# Autodesk Inventor assembly: ASSEMBLY_Outlet_channel_1
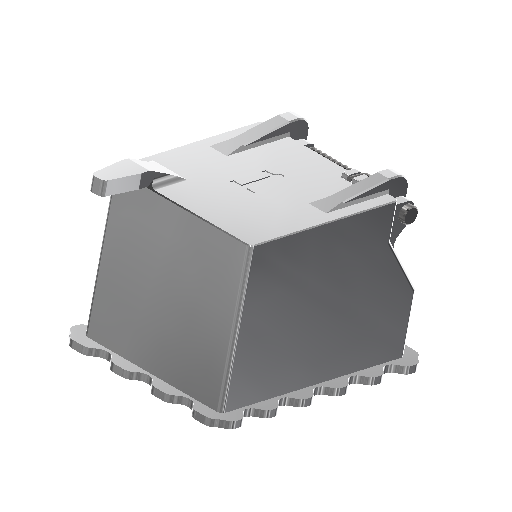
[picture p0: Inventor's stored thumbnail of the model, 512x512]
Saved by Autodesk Inventor 2025 (Build 290162010, 162A)
## iProperties
Created: 2018-09-15
Part Number: ASSEMBLY_Outlet_channel_1
Document SubType Name: Assembly
Designer: Andrzej
Mass: 26.9847 g
Surface Area: 139.625 cm^2
Volume: 9.56694 cm^3
Density: 2.82062 g/cm^3
Author: Andrzej
## Documents named in this file (5)
- D:\_ANDRZEJ_LACZEWSKI\_OTHER\MECH - My entry for the NASA Lunar Sampling System Design Challenge\MCAD\1_REV1\ASSEMBLY_MAIN_REVA\ASSEMBLY_Outlet_channel_1.iam
- D:\_ANDRZEJ_LACZEWSKI\_OTHER\MECH - My entry for the NASA Lunar Sampling System Design Challenge\MCAD\1_REV1\ASSEMBLY_MAIN_REVA\CNCT_STEEL_Outlet_door_hinge_pin.ipt
- D:\_ANDRZEJ_LACZEWSKI\_OTHER\MECH - My entry for the NASA Lunar Sampling System Design Challenge\MCAD\1_REV1\ASSEMBLY_MAIN_REVA\CNCM_ALU_Outlet_channel_door.ipt
- D:\_ANDRZEJ_LACZEWSKI\_OTHER\MECH - My entry for the NASA Lunar Sampling System Design Challenge\MCAD\1_REV1\ASSEMBLY_MAIN_REVA\CNCM_ALU_Outlet_channel.ipt
- D:\_ANDRZEJ_LACZEWSKI\_OTHER\MECH - My entry for the NASA Lunar Sampling System Design Challenge\MCAD\1_REV1\ASSEMBLY_MAIN_REVA\CUT_STEEL_Outlet_channel_door_spring.ipt
## Components (4 placed, 4 different names)
1. CNCM_ALU_Outlet_channel_door:1 — Mate:1, Mate:2, Mate:6, Angle:1
2. CNCM_ALU_Outlet_channel:1 — Mate:1, Mate:2, Mate:3, Mate:4, Angle:1
3. CNCT_STEEL_Outlet_door_hinge_pin:1 — Mate:3, Mate:4, Mate:5
4. CUT_STEEL_Outlet_channel_door_spring:1 — Mate:5, Mate:6
## Relationships (7: Mate 6, Angle 1)
- Mate:1: CNCM_ALU_Outlet_channel_door:1 ↔ CNCM_ALU_Outlet_channel:1
- Mate:2: CNCM_ALU_Outlet_channel_door:1 ↔ CNCM_ALU_Outlet_channel:1
- Mate:3: CNCM_ALU_Outlet_channel:1 ↔ CNCT_STEEL_Outlet_door_hinge_pin:1
- Mate:4: CNCM_ALU_Outlet_channel:1 ↔ CNCT_STEEL_Outlet_door_hinge_pin:1
- Mate:5: CNCT_STEEL_Outlet_door_hinge_pin:1 ↔ CUT_STEEL_Outlet_channel_door_spring:1
- Mate:6 (0.5 mm): CNCM_ALU_Outlet_channel_door:1 ↔ CUT_STEEL_Outlet_channel_door_spring:1
- Angle:1 (180 deg): CNCM_ALU_Outlet_channel_door:1 ↔ CNCM_ALU_Outlet_channel:1
